# Autodesk Inventor assembly: module_command
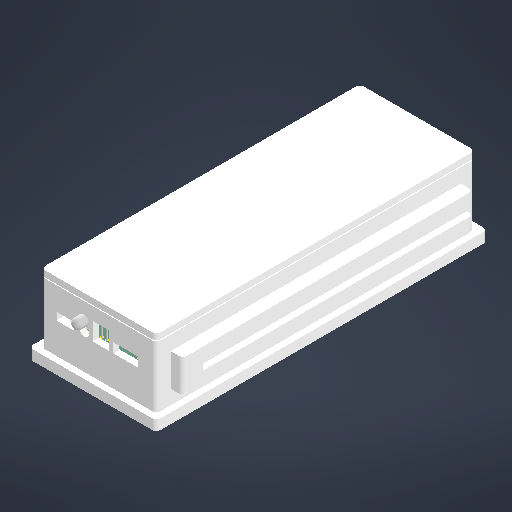
[picture p0: Inventor's stored thumbnail of the model, 512x512]
Saved by Autodesk Inventor 2025.2 (Build 292293000, 293)
## iProperties
Created: 2025-11-12
Part Number: module_command
Document SubType Name: Assembly
Designer: sam
Author: sam
## Documents named in this file (8)
- G:\projects\primary\regulated-irrigation-system\model\asm\module-command\module_command.iam
- G:\projects\primary\regulated-irrigation-system\model\asm\module-command\module_command.ipt
- G:\projects\primary\regulated-irrigation-system\model\asm\module-command\module-lid_command.ipt
- G:\projects\primary\regulated-irrigation-system\model\asm\electronic-components\pcb_command-module.iam
- G:\projects\primary\regulated-irrigation-system\model\asm\electronic-components\battery-5050100_4000.ipt
- G:\projects\primary\regulated-irrigation-system\model\asm\module-command\clip_pcb-command.ipt
- G:\projects\primary\regulated-irrigation-system\model\asm\electronic-components\boost-converter.ipt
- G:\projects\primary\regulated-irrigation-system\model\asm\electronic-components\charge-controller.ipt
## Components (8 placed, 7 different names)
1. module_command:1 — Mate:1, Mate:2, Mate:3, Mate:4, Mate:5, Mate:6, Mate:7, Mate:8, Mate:12, Mate:13, Mate:14, Mate:15, Mate:16, Mate:17, Mate:18, Mate:19, Mate:20
2. module-lid_command:1 — Mate:1, Mate:2
3. pcb_command-module:1 [sub-assembly] — Mate:9, Mate:10, Mate:11
4. battery-5050100_4000:1 — Mate:3, Mate:4, Mate:5
5. clip_pcb-command:1 — Mate:6, Mate:7, Mate:8, Mate:9, Mate:10, Mate:11
6. boost-converter:1 — Mate:15, Mate:16, Mate:17
7. boost-converter:2 — Mate:12, Mate:13, Mate:14
8. charge-controller:1 — Mate:18, Mate:19, Mate:20
## Relationships (20: Mate 20)
- Mate:1: module_command:1 ↔ module-lid_command:1
- Mate:2: module_command:1 ↔ module-lid_command:1
- Mate:3: module_command:1 ↔ battery-5050100_4000:1
- Mate:4 (0.2 mm): module_command:1 ↔ battery-5050100_4000:1
- Mate:5 (0.2 mm): module_command:1 ↔ battery-5050100_4000:1
- Mate:6: module_command:1 ↔ clip_pcb-command:1
- Mate:7 (0.2 mm): module_command:1 ↔ clip_pcb-command:1
- Mate:8 (0.2 mm): module_command:1 ↔ clip_pcb-command:1
- Mate:9 (0.2 mm): pcb_command-module:1 ↔ clip_pcb-command:1
- Mate:10: pcb_command-module:1 ↔ clip_pcb-command:1
- Mate:11 (0.2 mm): pcb_command-module:1 ↔ clip_pcb-command:1
- Mate:12 (0.2 mm): module_command:1 ↔ boost-converter:2
- Mate:13 (0.2 mm): module_command:1 ↔ boost-converter:2
- Mate:14: module_command:1 ↔ boost-converter:2
- Mate:15: module_command:1 ↔ boost-converter:1
- Mate:16 (0.2 mm): module_command:1 ↔ boost-converter:1
- Mate:17 (0.2 mm): module_command:1 ↔ boost-converter:1
- Mate:18 (0.2 mm): module_command:1 ↔ charge-controller:1
- Mate:19 (0.2 mm): module_command:1 ↔ charge-controller:1
- Mate:20: module_command:1 ↔ charge-controller:1
